# Autodesk Inventor assembly: Platform Sides Assembly
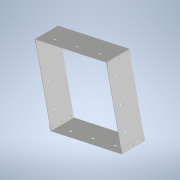
[picture p0: Inventor's stored thumbnail of the model, 180x180]
Saved by Autodesk Inventor 2020 (Build 240168000, 168)
## iProperties
Created: 2022-07-05
Part Number: Platform Sides Assembly
Document SubType Name: Assembly
Designer: karimi2
Author: karimi2
## Documents named in this file (3)
- C:\Users\karimi2\Documents\PROJECT\src\Platform Sides Assembly.iam
- C:\Users\karimi2\Documents\PROJECT\src\Platform side 1.ipt
- C:\Users\karimi2\Documents\PROJECT\src\Platform side 2.ipt
## Components (4 placed, 2 different names)
1. Platform side 1:1 — Mate:1, Rigid:1
2. Platform side 2:1 — Mate:1, Rigid:1, Mate:2, Rigid:2
3. Platform side 1:2 — Mate:2, Rigid:2, Mate:3, Rigid:3
4. Platform side 2:2 — Mate:3, Rigid:3
## Relationships (6: Mate 3, WeldJoint 3)
- Mate:1: Platform side 1:1 ↔ Platform side 2:1
- Rigid:1 [WeldJoint]: Platform side 1:1 ↔ Platform side 2:1
- Mate:2: Platform side 2:1 ↔ Platform side 1:2
- Rigid:2 [WeldJoint]: Platform side 2:1 ↔ Platform side 1:2
- Mate:3: Platform side 1:2 ↔ Platform side 2:2
- Rigid:3 [WeldJoint]: Platform side 1:2 ↔ Platform side 2:2
